# Autodesk Inventor assembly: Lenkung
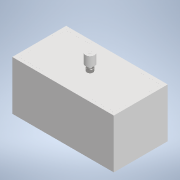
[picture p0: Inventor's stored thumbnail of the model, 180x180]
Saved by Autodesk Inventor 2020.3 (Build 243373010, 373A)
## iProperties
Created: 2020-11-28
Part Number: Lenkung
Document SubType Name: Assembly
Designer: Stefan
Author: Stefan
## Documents named in this file (13)
- D:\Stefan\Schule\HTL\Diplomarbeit\git\Inventor\Lenker\Lenkung.iam
- D:\Stefan\Schule\HTL\Diplomarbeit\git\Inventor\Lenker\Platte1.ipt
- D:\Stefan\Schule\HTL\Diplomarbeit\git\Inventor\Lenker\Platte2-Seite.ipt
- D:\Stefan\Schule\HTL\Diplomarbeit\git\Inventor\Lenker\Platte3-Seite.ipt
- D:\Stefan\Schule\HTL\Diplomarbeit\git\Inventor\Lenker\Platte4.ipt
- D:\Stefan\Schule\HTL\Diplomarbeit\git\Inventor\Lenker\Stange1Mitte.ipt
- D:\Stefan\Schule\HTL\Diplomarbeit\git\Inventor\Lenker\M4Gewindestange.ipt
- D:\Stefan\Schule\HTL\Diplomarbeit\git\Inventor\Lenker\Poti-RK09712_0-L15.ipt
- D:\Stefan\Schule\HTL\Diplomarbeit\git\Inventor\Lenker\StangePotiAdapter1.ipt
- D:\Stefan\Schule\HTL\Diplomarbeit\git\Inventor\Lenker\AdapterPoti2.ipt
- D:\Stefan\Schule\HTL\Diplomarbeit\git\Inventor\Lenker\PotiHalterungUnten.ipt
- C:\Users\Stefan\Documents\Inventor\Content Center Files\R2020\de-DE\DIN 705   B\DIN 705 - B10.ipt
- D:\Stefan\Schule\HTL\Diplomarbeit\git\Inventor\Lenker\stl\KoplungLenkerOben.ipt
## Components (16 placed, 12 different names)
1. Platte1:1 — Starr:1, Starr:2, Planar:1, Starr:19
2. Platte2-Seite:1 — Starr:2
3. Platte3-Seite:1 — Starr:1, Starr:17, Starr:18
4. Platte4:1 — Starr:16, Starr:18
5. Platte4:2 — Starr:15, Starr:17, Starr:20
6. Platte2-Seite:2 — Starr:19
7. Platte3-Seite:2 — Starr:20
8. Stange1Mitte:1 — Starr:7, Starr:8, Zylindrisch:1, Starr:21
9. M4Gewindestange:1 — Starr:7
10. Poti-RK09712_0-L15:1 — Drehbar:11, Starr:11
11. StangePotiAdapter1:1 — Starr:8, Starr:9
12. AdapterPoti2:1 — Starr:9, Drehbar:11
13. PotiHalterungUnten:1 — Planar:1, Starr:11
14. DIN 705 B B10:1 — Starr:15, Zylindrisch:1
15. DIN 705 B B10:2 — Starr:16
16. KoplungLenkerOben:1 — Starr:21
## Relationships (16: WeldJoint 13, RevoluteJoint 1, PlanarJoint 1, CylindricalJoint 1)
- Starr:1 [WeldJoint]: Platte1:1 ↔ Platte3-Seite:1
- Starr:2 [WeldJoint]: Platte1:1 ↔ Platte2-Seite:1
- Starr:7 [WeldJoint]: Stange1Mitte:1 ↔ M4Gewindestange:1
- Starr:8 [WeldJoint]: Stange1Mitte:1 ↔ StangePotiAdapter1:1
- Starr:9 [WeldJoint]: StangePotiAdapter1:1 ↔ AdapterPoti2:1
- Drehbar:11 [RevoluteJoint]: Poti-RK09712_0-L15:1 ↔ AdapterPoti2:1
- Planar:1: Platte1:1 ↔ PotiHalterungUnten:1
- Starr:11 [WeldJoint]: Poti-RK09712_0-L15:1 ↔ PotiHalterungUnten:1
- Starr:15 [WeldJoint]: Platte4:2 ↔ DIN 705 B B10:1
- Starr:16 [WeldJoint]: Platte4:1 ↔ DIN 705 B B10:2
- Starr:17 [WeldJoint]: Platte3-Seite:1 ↔ Platte4:2
- Starr:18 [WeldJoint]: Platte3-Seite:1 ↔ Platte4:1
- Zylindrisch:1 [CylindricalJoint]: Stange1Mitte:1 ↔ DIN 705 B B10:1
- Starr:19 [WeldJoint]: Platte1:1 ↔ Platte2-Seite:2
- Starr:20 [WeldJoint]: Platte4:2 ↔ Platte3-Seite:2
- Starr:21 [WeldJoint]: Stange1Mitte:1 ↔ KoplungLenkerOben:1
## Named parameters: HolzDicke = 12 mm
